# Autodesk Inventor assembly: Differential Swerve Drive V1
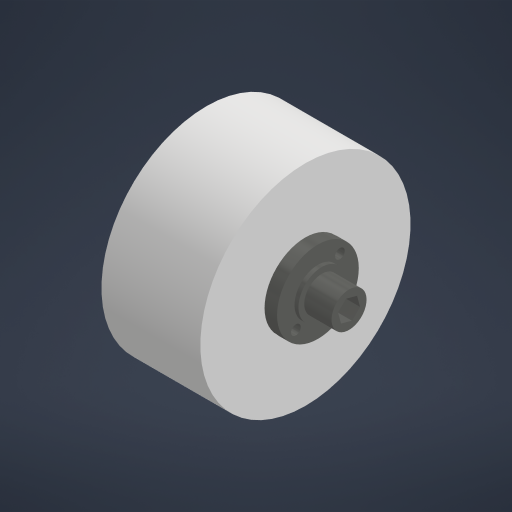
[picture p0: Inventor's stored thumbnail of the model, 512x512]
Saved by Autodesk Inventor 2023 (Build 270158000, 158)
## iProperties
Created: 2023-08-02
Part Number: Differential Swerve Drive V1
Document SubType Name: Assembly
Designer: izack
Author: izack
## Documents named in this file (3)
- D:\Robotics\Custom-Modules-CAD\Differential Swerve Drive V1\Differential Swerve Drive V1.iam
- D:\Robotics\Custom-Modules-CAD\Differential Swerve Drive V1\60mm_Grip_Wheel.ipt
- D:\Robotics\Custom-Modules-CAD\Differential Swerve Drive V1\Differential Swerve Drive Parts\High Strength Hub.ipt
## Components (3 placed, 2 different names)
1. 60mm_Grip_Wheel:1 — Mate:1, Mate:2, Mate:3, Mate:4, Mate:5, Mate:6
2. High Strength Hub:1 — Mate:4, Mate:5, Mate:6
3. High Strength Hub:2 — Mate:1, Mate:2, Mate:3
## Relationships (6: Mate 6)
- Mate:1: 60mm_Grip_Wheel:1 ↔ High Strength Hub:2
- Mate:2: 60mm_Grip_Wheel:1 ↔ High Strength Hub:2
- Mate:3: 60mm_Grip_Wheel:1 ↔ High Strength Hub:2
- Mate:4: 60mm_Grip_Wheel:1 ↔ High Strength Hub:1
- Mate:5: 60mm_Grip_Wheel:1 ↔ High Strength Hub:1
- Mate:6: 60mm_Grip_Wheel:1 ↔ High Strength Hub:1
